# Autodesk Inventor assembly: stay1_MIR
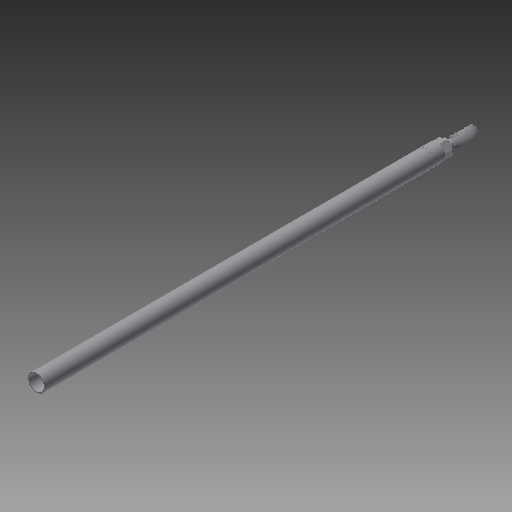
[picture p0: Inventor's stored thumbnail of the model, 512x512]
Saved by Autodesk Inventor 2018.2 (Build 222227000, 227)
## iProperties
Created: 2018-04-27
Part Number: stay1_MIR
Material: 一般
Document SubType Name: Assembly
Designer: formula
Author: ku_sk
## Documents named in this file (3)
- Z:\各班フォルダ\2018\ボディ\エアロ\Aero\KS-15\Rr.wing\parts\stay\stay1_MIR.iam
- Z:\各班フォルダ\2018\ボディ\エアロ\Aero\KS-15\Rr.wing\parts\stay\pipe_16mm_360mm_MIR.ipt
- Z:\各班フォルダ\2018\ボディ\エアロ\Aero\KS-15\Rr.wing\parts\stay\end\stay end_MIR.iam
## Components (2 placed, 2 different names)
1. pipe_16mm_360mm_MIR:1 — メイト:3, メイト:2, メイト:1, メイト:5, メイト:4
2. stay end_MIR:1 [sub-assembly] — メイト:5, メイト:4
## Relationships (5: Mate 5)
- メイト:3 [Mate]: pipe_16mm_360mm_MIR:1
- メイト:2 [Mate]: pipe_16mm_360mm_MIR:1
- メイト:1 [Mate]: pipe_16mm_360mm_MIR:1
- メイト:5 [Mate]: pipe_16mm_360mm_MIR:1 ↔ stay end_MIR:1
- メイト:4 [Mate]: pipe_16mm_360mm_MIR:1 ↔ stay end_MIR:1
